# Autodesk Inventor assembly: LER
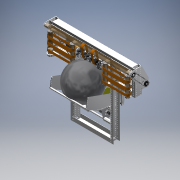
[picture p0: Inventor's stored thumbnail of the model, 180x180]
Saved by Autodesk Inventor 2019 (Build 230136000, 136)
## iProperties
Created: 2018-10-31
Part Number: LER
Document SubType Name: Assembly
Designer: woodk
Author: woodk
Revision Number: ANY
## Documents named in this file (14)
- E:\Shooter1678\Workspaces\Workspace\LER.iam
- E:\Shooter1678\Workspaces\Workspace\1678-16-A-0800.iam
- E:\Shooter1678\Workspaces\Workspace\bushing_.5.ipt
- E:\Shooter1678\Workspaces\Workspace\1678-16-P-0408.ipt
- E:\Shooter1678\Workspaces\Workspace\1678-16-P-0536.ipt
- E:\Shooter1678\Workspaces\Workspace\1678-16-P-0314-final.ipt
- E:\Shooter1678\Workspaces\Workspace\LER_shooter hood.iam
- E:\Shooter1678\Workspaces\Workspace\LER_intake.iam
- E:\Shooter1678\Workspaces\Workspace\Side arm outer.ipt
- E:\Shooter1678\Workspaces\Workspace\Side arm inner.ipt
- E:\Shooter1678\Workspaces\Workspace\Back brace.ipt
- E:\Shooter1678\Workspaces\Workspace\Boulder.ipt
- E:\Shooter1678\Workspaces\Workspace\Roller bracket.ipt
- E:\Shooter1678\Workspaces\Workspace\Roller bracket mirror.ipt
## Components (19 placed, 18 different names)
1. 1678-16-P-0401_118 — Insert:1, Insert:2, Insert:5, Insert:6, Insert:9, Insert:10, Insert:16, Insert:24, Insert:25, Insert:27, Insert:28, Insert:31, Insert:32
2. Mirror1678-16-P-0401_120 — Insert:3, Insert:4, Insert:7, Insert:8, Insert:11, Insert:12, Insert:17, Insert:22, Insert:23, Insert:29, Insert:30
3. 1678-16-A-0500_146 [sub-assembly] — Insert:9, Insert:10, Insert:11, Insert:12
4. 1678-16-A-0900_147 [sub-assembly] — Insert:19, Insert:20, Insert:21
5. 1678-16-A-0800_148 [sub-assembly] — Insert:26, Insert:27, Insert:28
6. bushing_.5_149 — Insert:18
7. bushing_.5_150 — Insert:17
8. bushing_.5_151 — Insert:16, Insert:19
9. bushing_.5_152 — Insert:14, Insert:15
10. 1678-16-P-0408_153 — Insert:14
11. 1678-16-P-0535_154 — Insert:29, Insert:30
12. Mirror1678-16-P-0535_155 — Insert:31, Insert:32
13. 1678-16-P-0536_156 — Insert:13
14. 1678-16-P-0409_157 — Insert:1, Insert:2, Insert:3, Insert:4
15. 1678-16-P-0314-final_166 — Insert:7, Insert:8, Insert:21
16. 1678-16-P-0314-final_167 — Insert:5, Insert:6, Insert:13, Insert:20, Insert:26
17. Side arm inner:1 — Insert:22, Insert:23, Insert:18
18. Side arm inner:2 — Insert:24, Insert:25, Insert:15
19. Boulder:1
## Relationships (32: Insert 32)
- Insert:1: 1678-16-P-0401_118 ↔ 1678-16-P-0409_157
- Insert:2: 1678-16-P-0401_118 ↔ 1678-16-P-0409_157
- Insert:3: Mirror1678-16-P-0401_120 ↔ 1678-16-P-0409_157
- Insert:4: Mirror1678-16-P-0401_120 ↔ 1678-16-P-0409_157
- Insert:5: 1678-16-P-0401_118 ↔ 1678-16-P-0314-final_167
- Insert:6: 1678-16-P-0401_118 ↔ 1678-16-P-0314-final_167
- Insert:7: Mirror1678-16-P-0401_120 ↔ 1678-16-P-0314-final_166
- Insert:8: Mirror1678-16-P-0401_120 ↔ 1678-16-P-0314-final_166
- Insert:9: 1678-16-P-0401_118 ↔ 1678-16-A-0500_146
- Insert:10: 1678-16-P-0401_118 ↔ 1678-16-A-0500_146
- Insert:11: Mirror1678-16-P-0401_120 ↔ 1678-16-A-0500_146
- Insert:12: Mirror1678-16-P-0401_120 ↔ 1678-16-A-0500_146
- Insert:13: 1678-16-P-0536_156 ↔ 1678-16-P-0314-final_167
- Insert:14 (-0.127 mm): bushing_.5_152 ↔ 1678-16-P-0408_153
- Insert:15: bushing_.5_152 ↔ Side arm inner:2
- Insert:16: 1678-16-P-0401_118 ↔ bushing_.5_151
- Insert:17: Mirror1678-16-P-0401_120 ↔ bushing_.5_150
- Insert:18: bushing_.5_149 ↔ Side arm inner:1
- Insert:19: 1678-16-A-0900_147 ↔ bushing_.5_151
- Insert:20: 1678-16-A-0900_147 ↔ 1678-16-P-0314-final_167
- Insert:21: 1678-16-A-0900_147 ↔ 1678-16-P-0314-final_166
- Insert:22: Mirror1678-16-P-0401_120 ↔ Side arm inner:1
- Insert:23: Mirror1678-16-P-0401_120 ↔ Side arm inner:1
- Insert:24: 1678-16-P-0401_118 ↔ Side arm inner:2
- Insert:25: 1678-16-P-0401_118 ↔ Side arm inner:2
- Insert:26: 1678-16-A-0800_148 ↔ 1678-16-P-0314-final_167
- Insert:27: 1678-16-P-0401_118 ↔ 1678-16-A-0800_148
- Insert:28: 1678-16-P-0401_118 ↔ 1678-16-A-0800_148
- Insert:29: Mirror1678-16-P-0401_120 ↔ 1678-16-P-0535_154
- Insert:30: Mirror1678-16-P-0401_120 ↔ 1678-16-P-0535_154
- Insert:31: 1678-16-P-0401_118 ↔ Mirror1678-16-P-0535_155
- Insert:32: 1678-16-P-0401_118 ↔ Mirror1678-16-P-0535_155
